# Autodesk Inventor assembly: edge tab
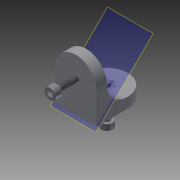
[picture p0: Inventor's stored thumbnail of the model, 180x180]
Saved by Autodesk Inventor 2014 (Build 180170000, 170)
## iProperties
Created: 2013-10-14
Part Number: edge tab
Document SubType Name: Assembly
Designer: employee
Author: employee
## Documents named in this file (4)
- \\GRISTLE\speco\GitHub\ConceptFORGE\Wally\edge tab.iam
- \\GRISTLE\speco\GitHub\ConceptFORGE\Wally\edge tab.ipt
- \\GRISTLE\speco\GitHub\ConceptFORGE\Wally\m3 nut.ipt
- \\GRISTLE\speco\GitHub\ConceptFORGE\Wally\M3x16.ipt
## Components (5 placed, 3 different names)
1. edge tab:1 — Insert:1, Insert:2, Angle:1, Angle:2, Insert:3, Insert:4
2. Hex Nut Metric M3 x 0.5:1 — Insert:1, Angle:1
3. Hex Nut Metric M3 x 0.5:2 — Insert:2, Angle:2
4. Forged Socket Head Cap Screw - Metric M3x0.5 x 16:1 — Insert:3
5. Forged Socket Head Cap Screw - Metric M3x0.5 x 16:2 — Insert:4
## Relationships (6: Insert 4, Angle 2)
- Insert:1: edge tab:1 ↔ Hex Nut Metric M3 x 0.5:1
- Insert:2: edge tab:1 ↔ Hex Nut Metric M3 x 0.5:2
- Angle:1 (0 deg): edge tab:1 ↔ Hex Nut Metric M3 x 0.5:1
- Angle:2 (0 deg): edge tab:1 ↔ Hex Nut Metric M3 x 0.5:2
- Insert:3 (9.5 mm): edge tab:1 ↔ Forged Socket Head Cap Screw - Metric M3x0.5 x 16:1
- Insert:4 (9.5 mm): edge tab:1 ↔ Forged Socket Head Cap Screw - Metric M3x0.5 x 16:2
